# Autodesk Inventor assembly: decoder_dual
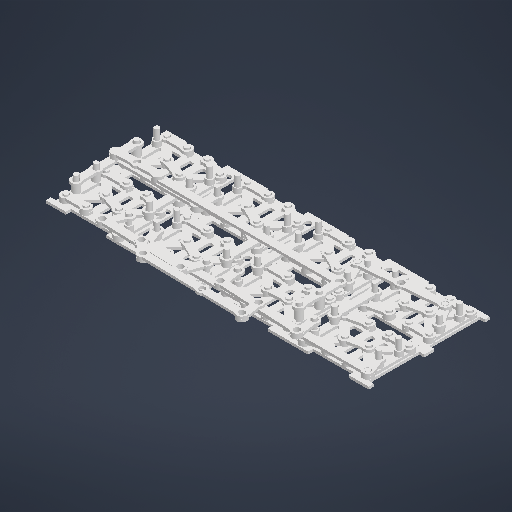
[picture p0: Inventor's stored thumbnail of the model, 512x512]
Saved by Autodesk Inventor 2025.4 (Build 294407000, 407)
## iProperties
Created: 2026-09-15
Part Number: decoder_dual
Document SubType Name: Assembly
Designer: User
Author: User
## Documents named in this file (17)
- G:\projects\primary\mechanical-computer\mechanics\gates\decoder_dual.iam
- G:\projects\primary\mechanical-computer\mechanics\lock\lock.iam
- G:\projects\primary\mechanical-computer\mechanics\links\link.ipt
- G:\projects\primary\mechanical-computer\mechanics\links\link\link-8.ipt
- G:\projects\primary\mechanical-computer\mechanics\links\link-1-turn-rigid\link-1-turn-rigid-8(_AS)4w-8l.ipt
- G:\projects\primary\mechanical-computer\mechanics\links\link-1-turn-rigid.ipt
- G:\projects\primary\mechanical-computer\mechanics\links\link\link-16.ipt
- G:\projects\primary\mechanical-computer\mechanics\links\link-split\link-split-16ab.ipt
- G:\projects\primary\mechanical-computer\mechanics\links\link-split.ipt
- G:\projects\primary\mechanical-computer\mechanics\links\link-split\link-split-8(_AS)5a-8(_AS)6b.ipt
- G:\projects\primary\mechanical-computer\mechanics\links\leveller.ipt
- G:\projects\primary\mechanical-computer\mechanics\links\leveller\leveller-2.ipt
- G:\projects\primary\mechanical-computer\mechanics\links\link-split\link-split-8(_AS)2ab.ipt
- G:\projects\primary\mechanical-computer\mechanics\links\link-split\link-split-8(_AS)3a-8(_AS)2b.ipt
- G:\projects\primary\mechanical-computer\mechanics\links\link-split\link-split-8ab-2endpins.ipt
- G:\projects\primary\mechanical-computer\mechanics\links\link-1-turn-rigid\link-1-turn-rigid-8(_AS)9w-8l.ipt
- G:\projects\primary\mechanical-computer\mechanics\links\link\link-8-1pin.ipt
## Components (37 placed, 13 different names)
1. link-1-turn-rigid-8(_AS)4w-8l:1 — Cylindrical:9, Cylindrical:10, Mate:12, Mate:21, Mate:23, Cylindrical:52
2. link-split-16ab:1 — Mate:20, Cylindrical:48, Cylindrical:50
3. link-split-8ab-2endpins:2 — Mate:22, Cylindrical:44, Cylindrical:45
4. link-1-turn-rigid-8(_AS)9w-8l:2 — Mate:23, Cylindrical:29, Cylindrical:30, Cylindrical:45
5. link-split-8(_AS)5a-8(_AS)6b:3 — Mate:25, Cylindrical:46, Cylindrical:47, Mate:48
6. lock:1 [sub-assembly] — Mate:1, Flush:1, Flush:2, Mate:3, Flush:5, Flush:6, Cylindrical:9, Cylindrical:10, Mate:12, Cylindrical:13, Mate:14, Mate:27, Mate:28, Mate:29, Mate:30, Cylindrical:53
7. lock:2 [sub-assembly] — Mate:1, Flush:1, Flush:2, Mate:7, Flush:13, Flush:14, Cylindrical:15, Mate:15, Cylindrical:32, Mate:26, Cylindrical:54
8. lock:3 [sub-assembly] — Mate:3, Flush:5, Flush:6, Cylindrical:14, Cylindrical:27, Mate:36, Mate:37
9. lock:4 [sub-assembly] — Cylindrical:12, Mate:13, Cylindrical:16
10. lock:5 [sub-assembly] — Mate:7, Flush:13, Flush:14, Cylindrical:17, Mate:16, Cylindrical:29, Cylindrical:30, Mate:32, Mate:33, Mate:34, Mate:35, Cylindrical:55
11. lock:6 [sub-assembly] — Cylindrical:19, Mate:17, Cylindrical:33, Mate:24, Cylindrical:56
12. lock:7 [sub-assembly] — Cylindrical:18, Mate:18, Cylindrical:51
13. lock:8 [sub-assembly] — Cylindrical:20, Mate:19, Cylindrical:49
14. leveller:1 — Mate:27, Mate:28
15. leveller:2 — Mate:29, Mate:30
16. leveller-2:3 — Mate:32, Mate:33
17. leveller-2:4 — Mate:34, Mate:35
18. leveller-2:5 — Mate:36, Mate:37
19. link-8-1pin:5 — Cylindrical:12, Mate:13, Cylindrical:52
20. link-8-1pin:12 — Mate:18, Cylindrical:50, Cylindrical:51
21. link-8-1pin:13 — Mate:19, Mate:20, Cylindrical:48, Cylindrical:49
22. link-8:14 — Cylindrical:27, Mate:21, Mate:22, Cylindrical:44
23. link-8-1pin:15 — Cylindrical:32, Mate:26, Cylindrical:47
24. link-8-1pin:16 — Cylindrical:33, Mate:24, Mate:25, Cylindrical:46
25. link-16:6 — Cylindrical:13, Cylindrical:14, Mate:14
26. link-16:7 — Cylindrical:15, Cylindrical:16, Mate:15
27. link-16:8 — Cylindrical:17, Cylindrical:18, Mate:16
28. link-16:9 — Cylindrical:19, Cylindrical:20, Mate:17
29. link-split-8(_AS)2ab:4 — Cylindrical:36, Cylindrical:38, Mate:38, Mate:39, Cylindrical:41, Mate:46
30. link-split-8(_AS)2ab:5 — Cylindrical:37, Cylindrical:39, Mate:40, Mate:41, Cylindrical:40, Mate:47
31. link-split-8(_AS)3a-8(_AS)2b:6 — Cylindrical:42, Cylindrical:43, Mate:44, Mate:45
32. link-8:21 — Cylindrical:41, Cylindrical:42, Mate:44, Mate:46
33. link-8:22 — Cylindrical:40, Cylindrical:43, Mate:45, Mate:47
34. link-8:18 — Cylindrical:36, Mate:39, Cylindrical:54
35. link-8:17 — Cylindrical:38, Mate:38, Cylindrical:53, Mate:48
36. link-8:19 — Cylindrical:39, Mate:40, Cylindrical:55
37. link-8:20 — Cylindrical:37, Mate:41, Cylindrical:56
## Relationships (92: Mate 41, CylindricalJoint 37, Flush 14)
- Mate:1: lock:1 ↔ lock:2
- Flush:1: lock:1 ↔ lock:2
- Flush:2: lock:1 ↔ lock:2
- [Mate]: lock:3 ↔ lock:4
- [Flush]: lock:3 ↔ lock:4
- [Flush]: lock:3 ↔ lock:4
- Mate:3: lock:1 ↔ lock:3
- Flush:5: lock:1 ↔ lock:3
- Flush:6: lock:1 ↔ lock:3
- [Mate]: lock:5 ↔ lock:6
- [Flush]: lock:5 ↔ lock:6
- [Flush]: lock:5 ↔ lock:6
- [Mate]: lock:7 ↔ lock:8
- [Flush]: lock:7 ↔ lock:8
- [Flush]: lock:7 ↔ lock:8
- [Mate]: lock:5 ↔ lock:7
- [Flush]: lock:5 ↔ lock:7
- [Flush]: lock:5 ↔ lock:7
- Mate:7: lock:2 ↔ lock:5
- Flush:13: lock:2 ↔ lock:5
- Flush:14: lock:2 ↔ lock:5
- Cylindrical:9: link-1-turn-rigid-8(_AS)4w-8l:1 ↔ lock:1
- Cylindrical:10: link-1-turn-rigid-8(_AS)4w-8l:1 ↔ lock:1
- Cylindrical:12: lock:4 ↔ link-8-1pin:5
- Mate:12 (1 mm): link-1-turn-rigid-8(_AS)4w-8l:1 ↔ lock:1
- Mate:13: lock:4 ↔ link-8-1pin:5
- Cylindrical:13: lock:1 ↔ link-16:6
- Cylindrical:14: lock:3 ↔ link-16:6
- Cylindrical:15: lock:2 ↔ link-16:7
- Cylindrical:16: lock:4 ↔ link-16:7
- Cylindrical:17: lock:5 ↔ link-16:8
- Cylindrical:18: lock:7 ↔ link-16:8
- Cylindrical:19: lock:6 ↔ link-16:9
- Cylindrical:20: lock:8 ↔ link-16:9
- Mate:14: lock:1 ↔ link-16:6
- Mate:15: lock:2 ↔ link-16:7
- Mate:16: lock:5 ↔ link-16:8
- Mate:17: lock:6 ↔ link-16:9
- Mate:18: lock:7 ↔ link-8-1pin:12
- Mate:19: lock:8 ↔ link-8-1pin:13
- Mate:20: link-split-16ab:1 ↔ link-8-1pin:13
- Cylindrical:27: lock:3 ↔ link-8:14
- Mate:21: link-1-turn-rigid-8(_AS)4w-8l:1 ↔ link-8:14
- Mate:22: link-split-8ab-2endpins:2 ↔ link-8:14
- Mate:23: link-1-turn-rigid-8(_AS)4w-8l:1 ↔ link-1-turn-rigid-8(_AS)9w-8l:2
- Cylindrical:29: link-1-turn-rigid-8(_AS)9w-8l:2 ↔ lock:5
- Cylindrical:30: link-1-turn-rigid-8(_AS)9w-8l:2 ↔ lock:5
- Cylindrical:32: lock:2 ↔ link-8-1pin:15
- Cylindrical:33: lock:6 ↔ link-8-1pin:16
- Mate:24: lock:6 ↔ link-8-1pin:16
- Mate:25: link-split-8(_AS)5a-8(_AS)6b:3 ↔ link-8-1pin:16
- Mate:26: lock:2 ↔ link-8-1pin:15
- Mate:27: lock:1 ↔ leveller:1
- Mate:28: lock:1 ↔ leveller:1
- Mate:29: lock:1 ↔ leveller:2
- Mate:30: lock:1 ↔ leveller:2
- Mate:32: lock:5 ↔ leveller-2:3
- Mate:33: lock:5 ↔ leveller-2:3
- Mate:34: lock:5 ↔ leveller-2:4
- Mate:35: lock:5 ↔ leveller-2:4
- Mate:36: lock:3 ↔ leveller-2:5
- Mate:37: lock:3 ↔ leveller-2:5
- Cylindrical:36: link-split-8(_AS)2ab:4 ↔ link-8:18
- Cylindrical:37: link-split-8(_AS)2ab:5 ↔ link-8:20
- Cylindrical:38: link-split-8(_AS)2ab:4 ↔ link-8:17
- Cylindrical:39: link-split-8(_AS)2ab:5 ↔ link-8:19
- Mate:38: link-split-8(_AS)2ab:4 ↔ link-8:17
- Mate:39: link-split-8(_AS)2ab:4 ↔ link-8:18
- Mate:40: link-split-8(_AS)2ab:5 ↔ link-8:19
- Mate:41: link-split-8(_AS)2ab:5 ↔ link-8:20
- Cylindrical:40: link-split-8(_AS)2ab:5 ↔ link-8:22
- Cylindrical:41: link-split-8(_AS)2ab:4 ↔ link-8:21
- Cylindrical:42: link-split-8(_AS)3a-8(_AS)2b:6 ↔ link-8:21
- Cylindrical:43: link-split-8(_AS)3a-8(_AS)2b:6 ↔ link-8:22
- Mate:44: link-split-8(_AS)3a-8(_AS)2b:6 ↔ link-8:21
- Mate:45: link-split-8(_AS)3a-8(_AS)2b:6 ↔ link-8:22
- Cylindrical:44: link-split-8ab-2endpins:2 ↔ link-8:14
- Cylindrical:45: link-split-8ab-2endpins:2 ↔ link-1-turn-rigid-8(_AS)9w-8l:2
- Cylindrical:46: link-split-8(_AS)5a-8(_AS)6b:3 ↔ link-8-1pin:16
- Cylindrical:47: link-split-8(_AS)5a-8(_AS)6b:3 ↔ link-8-1pin:15
- Cylindrical:48: link-split-16ab:1 ↔ link-8-1pin:13
- Cylindrical:49: lock:8 ↔ link-8-1pin:13
- Cylindrical:50: link-split-16ab:1 ↔ link-8-1pin:12
- Cylindrical:51: lock:7 ↔ link-8-1pin:12
- Cylindrical:52: link-1-turn-rigid-8(_AS)4w-8l:1 ↔ link-8-1pin:5
- Mate:46: link-split-8(_AS)2ab:4 ↔ link-8:21
- Mate:47: link-split-8(_AS)2ab:5 ↔ link-8:22
- Cylindrical:53: lock:1 ↔ link-8:17
- Cylindrical:54: lock:2 ↔ link-8:18
- Cylindrical:55: lock:5 ↔ link-8:19
- Cylindrical:56: lock:6 ↔ link-8:20
- Mate:48: link-split-8(_AS)5a-8(_AS)6b:3 ↔ link-8:17
## Named parameters: d34_d31 = 0 mm, d35_d32 = 0 mm, d36_d33 = 0 mm, d46_d43 = 0 mm, d47_d44 = 0 mm, d48_d45 = 0 mm, d49_d31 = 0 mm, d50_d32 = 0 mm, d51_d33 = 0 mm, d52_d34_d31 = 0 mm, d53_d35_d32 = 0 mm, d54_d36_d33 = 0 mm
